# Autodesk Inventor assembly: Assembly - 4
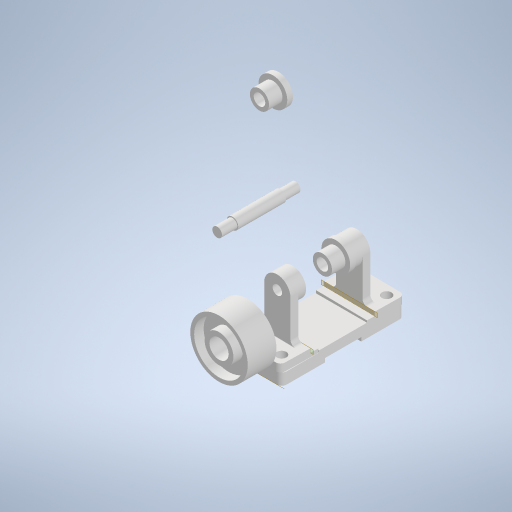
[picture p0: Inventor's stored thumbnail of the model, 512x512]
Saved by Autodesk Inventor 2024 (Build 280153000, 153)
## iProperties
Created: 2024-04-20
Part Number: Assembly - 4
Document SubType Name: Assembly
Designer: Ricsi
Author: Ricsi
## Documents named in this file (6)
- D:\Dokumentumok\VTS\Gépelemek 1\4\Assembly - 4.iam
- D:\Dokumentumok\VTS\Gépelemek 1\4\4 - Part 1.ipt
- D:\Dokumentumok\VTS\Gépelemek 1\4\4 - Part 2.ipt
- D:\Dokumentumok\VTS\Gépelemek 1\4\4 - Part 3.ipt
- D:\Dokumentumok\VTS\Gépelemek 1\4\4 - Part 4.ipt
- D:\Dokumentumok\VTS\Gépelemek 1\4\4 - Part 5.ipt
## Components (7 placed, 5 different names)
1. 4 - Part 1:1 — Mate:3, Mate:4
2. 4 - Part 1:2 — Mate:2
3. 4 - Part 2:1 — Mate:4
4. 4 - Part 2:2
5. 4 - Part 3:1
6. 4 - Part 4:1
7. 4 - Part 5:1 — Mate:1, Mate:2, Mate:3
## Relationships (4: Mate 4)
- Mate:1: 4 - Part 5:1
- Mate:2: 4 - Part 1:2 ↔ 4 - Part 5:1
- Mate:3: 4 - Part 1:1 ↔ 4 - Part 5:1
- Mate:4: 4 - Part 1:1 ↔ 4 - Part 2:1
